# Autodesk Inventor assembly: Assembly3
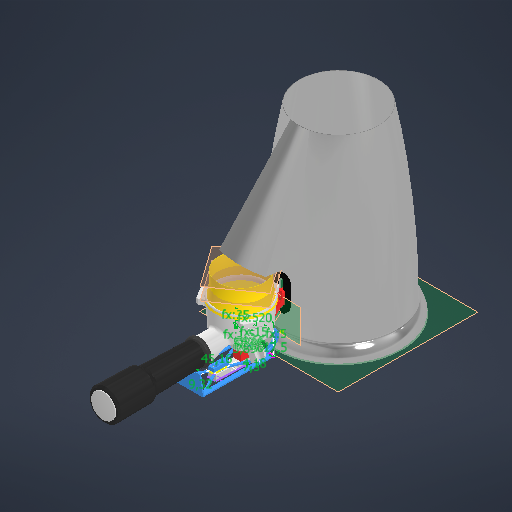
[picture p0: Inventor's stored thumbnail of the model, 512x512]
Saved by Autodesk Inventor 2026 (Build 300175000, 175)
## iProperties
Created: 2025-04-29
Part Number: Assembly3
Document SubType Name: Assembly
Designer: Paul Juschitz
Author: Paul Juschitz
## Documents named in this file (7)
- C:\Users\Paul Juschitz\Documents\private\m5_GBW_mod\M5_GBW_mod\CAD\Assembly3.iam
- C:\Users\Paul Juschitz\Documents\private\m5_GBW_mod\M5_GBW_mod\CAD\load_cell.ipt
- C:\Users\Paul Juschitz\Documents\private\m5_GBW_mod\M5_GBW_mod\CAD\m2m_shell.ipt
- C:\Users\Paul Juschitz\Documents\private\m5_GBW_mod\M5_GBW_mod\CAD\mock_dosing_funnel.ipt
- C:\Users\Paul Juschitz\Documents\private\m5_GBW_mod\M5_GBW_mod\CAD\load_cell_bracket.ipt
- C:\Users\Paul Juschitz\Documents\private\m5_GBW_mod\M5_GBW_mod\CAD\my_portafilter_holder_7.ipt
- C:\Users\Paul Juschitz\Documents\private\m5_GBW_mod\M5_GBW_mod\CAD\downloads\portafilter\BES870XL Portafilter\BES870XL Portafilter\BES870XL Portafilter_assembled.iam
## Components (6 placed, 6 different names)
1. load_cell:1 — Cylindrical:2, Cylindrical:3, Mate:3, Cylindrical:4, Cylindrical:5, Mate:4, Mate:5, Cylindrical:6, Mate:6
2. m2m_shell:1 — Mate:1, Flush:1, Angle:1, Angle:2, Tangent:3
3. BES870XL Portafilter_assembled:1 [sub-assembly] — Flush:1, Tangent:1, Tangent:2, Cylindrical:1, Angle:2, Mate:2
4. mock_dosing_funnel:1 — Cylindrical:1, Mate:2
5. my_portafilter_holder_7:1 — Mate:1, Tangent:1, Tangent:2, Angle:1, Cylindrical:2, Cylindrical:3, Mate:3, Mate:5, Cylindrical:6
6. load_cell_bracket:1 — Cylindrical:4, Cylindrical:5, Mate:4, Tangent:3, Mate:6
## Relationships (18: Mate 6, CylindricalJoint 6, Tangent 3, Angle 2, Flush 1)
- Mate:1: m2m_shell:1 ↔ my_portafilter_holder_7:1
- Flush:1: m2m_shell:1 ↔ BES870XL Portafilter_assembled:1
- Tangent:1: BES870XL Portafilter_assembled:1 ↔ my_portafilter_holder_7:1
- Tangent:2: BES870XL Portafilter_assembled:1 ↔ my_portafilter_holder_7:1
- Cylindrical:1: BES870XL Portafilter_assembled:1 ↔ mock_dosing_funnel:1
- Angle:1 (0 deg): m2m_shell:1 ↔ my_portafilter_holder_7:1
- Angle:2 (0 deg): m2m_shell:1 ↔ BES870XL Portafilter_assembled:1
- Mate:2: BES870XL Portafilter_assembled:1 ↔ mock_dosing_funnel:1
- Cylindrical:2: load_cell:1 ↔ my_portafilter_holder_7:1
- Cylindrical:3: load_cell:1 ↔ my_portafilter_holder_7:1
- Mate:3: load_cell:1 ↔ my_portafilter_holder_7:1
- Cylindrical:4: load_cell:1 ↔ load_cell_bracket:1
- Cylindrical:5: load_cell:1 ↔ load_cell_bracket:1
- Mate:4: load_cell:1 ↔ load_cell_bracket:1
- Mate:5: load_cell:1 ↔ my_portafilter_holder_7:1
- Cylindrical:6: load_cell:1 ↔ my_portafilter_holder_7:1
- Tangent:3: m2m_shell:1 ↔ load_cell_bracket:1
- Mate:6: load_cell:1 ↔ load_cell_bracket:1
